# Autodesk Inventor assembly: Assembly1
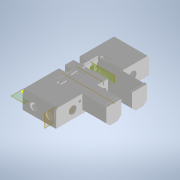
[picture p0: Inventor's stored thumbnail of the model, 180x180]
Saved by Autodesk Inventor 2022 (Build 260153000, 153)
## iProperties
Created: 2020-04-25
Part Number: Assembly1
Document SubType Name: Assembly
Designer: Martijn
Author: Martijn
## Documents named in this file (5)
- D:\phd\cad files\25 04 20 tiepieLCR case - Copy\Assembly1.iam
- D:\phd\cad files\25 04 20 tiepieLCR case - Copy\Part1.ipt
- D:\phd\cad files\25 04 20 tiepieLCR case - Copy\Part2.ipt
- D:\phd\cad files\25 04 20 tiepieLCR case - Copy\Part3.ipt
- D:\phd\cad files\25 04 20 tiepieLCR case - Copy\Part4.ipt
## Components (4 placed, 4 different names)
1. Part1:1 — Mate:1, Flush:1, Flush:2, Mate:2, Flush:3, Flush:4
2. Part2:1 — Mate:1, Flush:1, Flush:2, Mate:3, Mate:4
3. Part3:1 — Mate:2, Flush:3, Flush:4
4. Part4:1 — Mate:3, Mate:4
## Relationships (8: Mate 4, Flush 4)
- Mate:1: Part1:1 ↔ Part2:1
- Flush:1: Part1:1 ↔ Part2:1
- Flush:2: Part1:1 ↔ Part2:1
- Mate:2: Part1:1 ↔ Part3:1
- Flush:3: Part1:1 ↔ Part3:1
- Flush:4: Part1:1 ↔ Part3:1
- Mate:3: Part2:1 ↔ Part4:1
- Mate:4: Part2:1 ↔ Part4:1
